# Autodesk Inventor assembly: assembly_holder
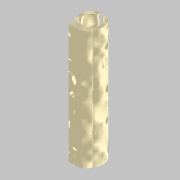
[picture p0: Inventor's stored thumbnail of the model, 180x180]
Saved by Autodesk Inventor 2021 (Build 250183000, 183)
## iProperties
Created: 2021-06-02
Part Number: assembly_holder
Document SubType Name: Assembly
Designer: Watchdog
Author: Watchdog
## Documents named in this file (3)
- C:\Users\Watchdog\OneDrive - Flinders\Advn Mech Design Shared\6_Development\2_Design\inventor\securing_mechanism\securingMechanism_variant_vertical_x\assembly_holder.iam
- C:\Users\Watchdog\OneDrive - Flinders\Advn Mech Design Shared\6_Development\2_Design\inventor\securing_mechanism\securingMechanism_variant_vertical_x\holder.ipt
- C:\Users\Watchdog\OneDrive - Flinders\Advn Mech Design Shared\6_Development\2_Design\inventor\securing_mechanism\securingMechanism_variant_vertical_x\holder_clamp.ipt
## Components (2 placed, 2 different names)
1. holder:1 — Mate:1, Flush:1, Mate:3, Flush:2
2. holder_clamp:1 — Flush:1
## Relationships (4: Mate 2, Flush 2)
- Mate:1: holder:1
- Flush:1: holder:1 ↔ holder_clamp:1
- Mate:3: holder:1
- Flush:2: holder:1
